# Autodesk Inventor assembly: Emblem
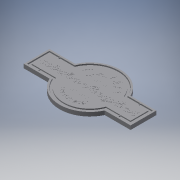
[picture p0: Inventor's stored thumbnail of the model, 180x180]
Saved by Autodesk Inventor 2019.3 (Build 233278000, 278)
## iProperties
Created: 2020-09-20
Part Number: Emblem
Material: Generisch
Document SubType Name: Assembly
Designer: Nicolas Frick
Author: Nicolas Frick
## Documents named in this file (3)
- C:\Users\Nicolas Frick\Sync\OneDrive\airhockeybot\mechanical_design\inventor\Emblem.iam
- C:\Users\Nicolas Frick\Sync\OneDrive\airhockeybot\mechanical_design\inventor\Emblem.ipt
- C:\Users\Nicolas Frick\Sync\OneDrive\airhockeybot\mechanical_design\inventor\Emblem_mask.ipt
## Components (2 placed, 2 different names)
1. Emblem:1 — Passend:1, Passend:3, Passend:4, Passend:5, Fluchtend:1, Fluchtend:2
2. Emblem_mask:1 — Passend:3, Passend:4, Passend:5
## Relationships (6: Mate 4, Flush 2)
- Passend:1 [Mate]: Emblem:1
- Passend:3 [Mate]: Emblem:1 ↔ Emblem_mask:1
- Passend:4 [Mate]: Emblem:1 ↔ Emblem_mask:1
- Passend:5 [Mate]: Emblem:1 ↔ Emblem_mask:1
- Fluchtend:1 [Flush]: Emblem:1
- Fluchtend:2 [Flush]: Emblem:1
